# Autodesk Inventor assembly: Motor_Bracket
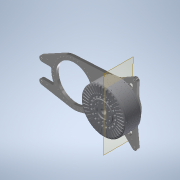
[picture p0: Inventor's stored thumbnail of the model, 180x180]
Saved by Autodesk Inventor 2021 (Build 250183000, 183)
## iProperties
Created: 2020-10-27
Part Number: Motor_Bracket
Document SubType Name: Assembly
Designer: PhotonUser
Quantity: 1
Author: PhotonUser
## Documents named in this file (3)
- D:\PhotonUser\Downloads\Assembly Files-20201026T232416Z-001\Assembly Files\Motor_Bracket.iam
- D:\PhotonUser\Downloads\Assembly Files-20201026T232416Z-001\Assembly Files\208_lc_resolver.iam
- D:\PhotonUser\Downloads\Assembly Files-20201026T232416Z-001\Assembly Files\Plate.ipt
## Components (2 placed, 2 different names)
1. Plate:1 — Insert:1, Insert:2
2. 208_lc_resolver:1 [sub-assembly] — Insert:1, Insert:2
## Relationships (2: Insert 2)
- Insert:1: Plate:1 ↔ 208_lc_resolver:1
- Insert:2: Plate:1 ↔ 208_lc_resolver:1
